# Autodesk Inventor assembly: 000-belt_liner_v1
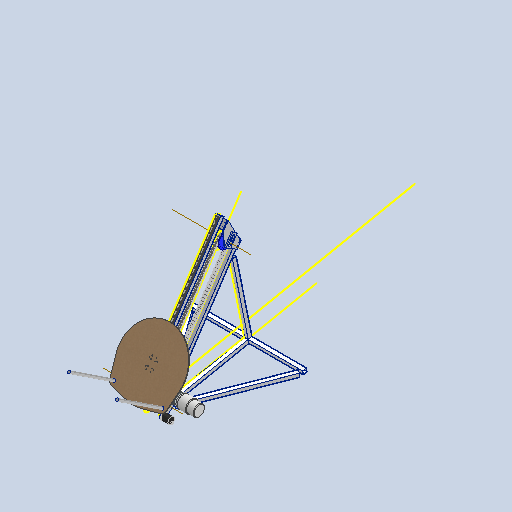
[picture p0: Inventor's stored thumbnail of the model, 512x512]
Saved by Autodesk Inventor 2025.1 (Build 291241000, 241)
## iProperties
Created: 2024-12-08
Part Number: 000-belt_liner_v1
Document SubType Name: Assembly
Designer: haruy
Author: haruy
## Documents named in this file (26)
- C:\Users\haruy\Documents\ロボコン\NHK2025\cad\nagahisa\belt_liner\000-belt_liner_v1.iam
- C:\Users\haruy\Documents\ロボコン\NHK2025\cad\nagahisa\belt_liner\belt_liner_v1_ASP_Base.ipt
- C:\Users\haruy\Documents\ロボコン\NHK2025\cad\nagahisa\belt_liner\SSE2B-MX10-455.iam
- C:\Users\haruy\Documents\ロボコン\NHK2025\cad\nagahisa\belt_liner\belt_liner_v1_Plate_1.ipt
- C:\Users\haruy\Documents\ロボコン\NHK2025\cad\nagahisa\belt_liner\belt_liner_v1_Plate_2.ipt
- C:\Users\haruy\Documents\ロボコン\NHK2025\cad\nagahisa\belt_liner\belt_liner_v1_Plate_3.ipt
- C:\Users\haruy\Documents\ロボコン\NHK2025\cad\000_parts\ベアリング\10\bear_10_15_sn.ipt
- C:\Users\haruy\Documents\ロボコン\NHK2025\cad\nagahisa\belt_liner\belt_liner_v1_shaft_spesa-25.ipt
- C:\Users\haruy\Documents\ロボコン\NHK2025\cad\nagahisa\belt_liner\belt_liner_v1_Plate_4.ipt
- C:\Users\haruy\Documents\ロボコン\NHK2025\cad\nagahisa\belt_liner\belt_liner_v1_Plate_5.ipt
- C:\Users\haruy\Documents\ロボコン\NHK2025\cad\000_parts\モーター\RS-775GM_004GH.iam
- C:\Users\haruy\Documents\ロボコン\NHK2025\cad\000_parts\エンコーダー\encoder v2.ipt
- C:\Users\haruy\Documents\ロボコン\NHK2025\cad\nagahisa\belt_liner\belt_liner_v1_Plate_6.ipt
- C:\Users\haruy\Documents\ロボコン\NHK2025\cad\nagahisa\belt_liner\belt_liner_v1_Plate_7.ipt
- C:\Users\haruy\Documents\ロボコン\NHK2025\cad\nagahisa\belt_liner\belt_liner_v1_Plate_8.ipt
- C:\Users\haruy\Documents\ロボコン\NHK2025\cad\nagahisa\belt_liner\belt_liner_v1_Plate_9.ipt
- C:\Users\haruy\Documents\ロボコン\NHK2025\cad\nagahisa\belt_liner\000-belt_liner_v1\デザイン アクセラレータ\歯付きベルト伝達1.iam
- C:\Users\haruy\Documents\ロボコン\NHK2025\cad\nagahisa\belt_liner\belt_liner_v1_shaft-54.ipt
- C:\Users\haruy\Documents\ロボコン\NHK2025\cad\nagahisa\belt_liner\SCSWJ10-6.iam
- C:\Users\haruy\Documents\ロボコン\NHK2025\cad\nagahisa\belt_liner\belt_liner_v1_shaft-84.ipt
- C:\Users\haruy\Documents\ロボコン\NHK2025\cad\nagahisa\belt_liner\000-belt_liner_v1\デザイン アクセラレータ\平歯車1.iam
- C:\Users\haruy\Documents\ロボコン\NHK2025\cad\nagahisa\belt_liner\000-belt_liner_v1\デザイン アクセラレータ\平歯車1_MIR.iam
- C:\Users\haruy\Documents\ロボコン\NHK2025\cad\nagahisa\belt_liner\belt_liner_v1_3DP_spesa-1.ipt
- C:\Users\haruy\Documents\ロボコン\NHK2025\cad\nagahisa\belt_liner\belt_liner_v1_3DP_spesa-2.ipt
- C:\Users\haruy\Documents\ロボコン\NHK2025\cad\nagahisa\belt_liner\belt_liner_v1_MDF_throw_plate.ipt
- C:\Users\haruy\Documents\ロボコン\NHK2025\cad\nagahisa\belt_liner\belt_liner_v1_shaft-200.ipt
## Components (44 placed, 25 different names)
1. belt_liner_v1_ASP_Base:1 — 挿入:1, 挿入:2, 挿入:3, 挿入:4, 挿入:5, 挿入:6, 挿入:28, 挿入:29, 挿入:30, 挿入:31, フラッシュ:1
2. SSE2B-MX10-455:1 [sub-assembly] — 挿入:1, 挿入:2, 挿入:51, 挿入:52
3. belt_liner_v1_Plate_1:1 — 挿入:3, 挿入:4
4. belt_liner_v1_Plate_2:1 — 挿入:5, 挿入:6, 挿入:7, 挿入:8, 挿入:9, 挿入:10
5. belt_liner_v1_Plate_3:1 — 挿入:7, 挿入:8, 挿入:12, 挿入:13, 挿入:14, 挿入:15, 挿入:16
6. belt_liner_v1_Plate_3:2 — 挿入:9, 挿入:10, 挿入:11, 挿入:19, 挿入:20, 挿入:21, 挿入:22
7. bear_10_15_sn:1 — 挿入:11
8. bear_10_15_sn:2 — 挿入:12, 挿入:50
9. belt_liner_v1_shaft_spesa-25:1 — 挿入:13, 挿入:17
10. belt_liner_v1_shaft_spesa-25:2 — 挿入:14, 挿入:18
11. belt_liner_v1_shaft_spesa-25:3 — 挿入:15
12. belt_liner_v1_shaft_spesa-25:4 — 挿入:16
13. belt_liner_v1_Plate_4:1 — 挿入:17, 挿入:18, 挿入:25, 挿入:27
14. belt_liner_v1_shaft_spesa-25:5 — 挿入:19, 挿入:24
15. belt_liner_v1_shaft_spesa-25:6 — 挿入:21
16. belt_liner_v1_shaft_spesa-25:7 — 挿入:20, 挿入:23
17. belt_liner_v1_shaft_spesa-25:8 — 挿入:22
18. belt_liner_v1_Plate_5:1 — 挿入:23, 挿入:24, 挿入:26
19. RS-775GM_004GH:1 [sub-assembly] — 挿入:25
20. RS-775GM_004GH:2 [sub-assembly] — 挿入:26, メイト:3
21. encoder v2:1 — 挿入:27
22. belt_liner_v1_Plate_6:1 — 挿入:28, 挿入:29, 挿入:32, 挿入:34, 挿入:35
23. belt_liner_v1_Plate_7:1 — 挿入:30, 挿入:31, 挿入:33
24. belt_liner_v1_Plate_8:1 — 挿入:32, 挿入:33, 挿入:36, 挿入:37
25. belt_liner_v1_Plate_8:2 — 挿入:34, 挿入:35, 挿入:38, 挿入:39
26. belt_liner_v1_Plate_9:1 — 挿入:38, 挿入:39
27. belt_liner_v1_Plate_9:2 — 挿入:36, 挿入:37
28. 歯付きベルト伝達:1 [sub-assembly] — 挿入:40, 挿入:41, 挿入:43, 挿入:49
29. bear_10_15_sn:3 — 挿入:40, 挿入:42, 挿入:47
30. bear_10_15_sn:4 — 挿入:41, 挿入:48
31. belt_liner_v1_shaft-54:1 — 挿入:42
32. SCSWJ10-6:1 [sub-assembly] — 挿入:43, 挿入:44
33. belt_liner_v1_shaft-84:1 — 挿入:44, 挿入:45, 挿入:46, メイト:1
34. SCSWJ10-6:2 [sub-assembly] — 挿入:45
35. SCSWJ10-6:3 [sub-assembly] — 挿入:46, メイト:2
36. 平歯車:1 [sub-assembly] — メイト:1, メイト:2, メイト:3
37. 平歯車1_MIR:1 [sub-assembly]
38. belt_liner_v1_3DP_spesa-1:1 — 挿入:47
39. belt_liner_v1_3DP_spesa-1:2 — 挿入:48
40. belt_liner_v1_3DP_spesa-1:3 — 挿入:49
41. belt_liner_v1_3DP_spesa-2:1 — 挿入:50
42. belt_liner_v1_MDF_throw_plate:1 — 挿入:51, 挿入:52, 挿入:53, 挿入:54
43. belt_liner_v1_shaft-200:1 — 挿入:54
44. belt_liner_v1_shaft-200:2 — 挿入:53
## Relationships (58: Insert 54, Mate 3, Flush 1)
- 挿入:1 [Insert]: belt_liner_v1_ASP_Base:1 ↔ SSE2B-MX10-455:1
- 挿入:2 [Insert]: belt_liner_v1_ASP_Base:1 ↔ SSE2B-MX10-455:1
- 挿入:3 [Insert]: belt_liner_v1_ASP_Base:1 ↔ belt_liner_v1_Plate_1:1
- 挿入:4 [Insert]: belt_liner_v1_ASP_Base:1 ↔ belt_liner_v1_Plate_1:1
- 挿入:5 [Insert]: belt_liner_v1_ASP_Base:1 ↔ belt_liner_v1_Plate_2:1
- 挿入:6 [Insert]: belt_liner_v1_ASP_Base:1 ↔ belt_liner_v1_Plate_2:1
- 挿入:7 [Insert]: belt_liner_v1_Plate_2:1 ↔ belt_liner_v1_Plate_3:1
- 挿入:8 [Insert]: belt_liner_v1_Plate_2:1 ↔ belt_liner_v1_Plate_3:1
- 挿入:9 [Insert]: belt_liner_v1_Plate_2:1 ↔ belt_liner_v1_Plate_3:2
- 挿入:10 [Insert]: belt_liner_v1_Plate_2:1 ↔ belt_liner_v1_Plate_3:2
- 挿入:11 [Insert]: belt_liner_v1_Plate_3:2 ↔ bear_10_15_sn:1
- 挿入:12 [Insert]: belt_liner_v1_Plate_3:1 ↔ bear_10_15_sn:2
- 挿入:13 [Insert]: belt_liner_v1_Plate_3:1 ↔ belt_liner_v1_shaft_spesa-25:1
- 挿入:14 [Insert]: belt_liner_v1_Plate_3:1 ↔ belt_liner_v1_shaft_spesa-25:2
- 挿入:15 [Insert]: belt_liner_v1_Plate_3:1 ↔ belt_liner_v1_shaft_spesa-25:3
- 挿入:16 [Insert]: belt_liner_v1_Plate_3:1 ↔ belt_liner_v1_shaft_spesa-25:4
- 挿入:17 [Insert]: belt_liner_v1_shaft_spesa-25:1 ↔ belt_liner_v1_Plate_4:1
- 挿入:18 [Insert]: belt_liner_v1_shaft_spesa-25:2 ↔ belt_liner_v1_Plate_4:1
- 挿入:19 [Insert]: belt_liner_v1_Plate_3:2 ↔ belt_liner_v1_shaft_spesa-25:5
- 挿入:20 [Insert]: belt_liner_v1_Plate_3:2 ↔ belt_liner_v1_shaft_spesa-25:7
- 挿入:21 [Insert]: belt_liner_v1_Plate_3:2 ↔ belt_liner_v1_shaft_spesa-25:6
- 挿入:22 [Insert]: belt_liner_v1_Plate_3:2 ↔ belt_liner_v1_shaft_spesa-25:8
- 挿入:23 [Insert]: belt_liner_v1_shaft_spesa-25:7 ↔ belt_liner_v1_Plate_5:1
- 挿入:24 [Insert]: belt_liner_v1_shaft_spesa-25:5 ↔ belt_liner_v1_Plate_5:1
- 挿入:25 [Insert]: belt_liner_v1_Plate_4:1 ↔ RS-775GM_004GH:1
- 挿入:26 [Insert]: belt_liner_v1_Plate_5:1 ↔ RS-775GM_004GH:2
- 挿入:27 [Insert]: belt_liner_v1_Plate_4:1 ↔ encoder v2:1
- 挿入:28 [Insert]: belt_liner_v1_ASP_Base:1 ↔ belt_liner_v1_Plate_6:1
- 挿入:29 [Insert]: belt_liner_v1_ASP_Base:1 ↔ belt_liner_v1_Plate_6:1
- 挿入:30 [Insert]: belt_liner_v1_ASP_Base:1 ↔ belt_liner_v1_Plate_7:1
- 挿入:31 [Insert]: belt_liner_v1_ASP_Base:1 ↔ belt_liner_v1_Plate_7:1
- 挿入:32 [Insert]: belt_liner_v1_Plate_6:1 ↔ belt_liner_v1_Plate_8:1
- 挿入:33 [Insert]: belt_liner_v1_Plate_7:1 ↔ belt_liner_v1_Plate_8:1
- 挿入:34 [Insert]: belt_liner_v1_Plate_6:1 ↔ belt_liner_v1_Plate_8:2
- 挿入:35 [Insert]: belt_liner_v1_Plate_6:1 ↔ belt_liner_v1_Plate_8:2
- 挿入:36 [Insert]: belt_liner_v1_Plate_8:1 ↔ belt_liner_v1_Plate_9:2
- 挿入:37 [Insert]: belt_liner_v1_Plate_8:1 ↔ belt_liner_v1_Plate_9:2
- 挿入:38 [Insert]: belt_liner_v1_Plate_8:2 ↔ belt_liner_v1_Plate_9:1
- 挿入:39 [Insert]: belt_liner_v1_Plate_8:2 ↔ belt_liner_v1_Plate_9:1
- フラッシュ:1 [Flush] (-7.5 mm): belt_liner_v1_ASP_Base:1
- 挿入:40 [Insert]: 歯付きベルト伝達:1 ↔ bear_10_15_sn:3
- 挿入:41 [Insert]: 歯付きベルト伝達:1 ↔ bear_10_15_sn:4
- 挿入:42 [Insert] (-16.5 mm): bear_10_15_sn:3 ↔ belt_liner_v1_shaft-54:1
- 挿入:43 [Insert]: 歯付きベルト伝達:1 ↔ SCSWJ10-6:1
- 挿入:44 [Insert] (-26.5 mm): SCSWJ10-6:1 ↔ belt_liner_v1_shaft-84:1
- 挿入:45 [Insert]: belt_liner_v1_shaft-84:1 ↔ SCSWJ10-6:2
- 挿入:46 [Insert]: belt_liner_v1_shaft-84:1 ↔ SCSWJ10-6:3
- メイト:1 [Mate]: belt_liner_v1_shaft-84:1 ↔ 平歯車:1
- メイト:2 [Mate]: SCSWJ10-6:3 ↔ 平歯車:1
- メイト:3 [Mate]: RS-775GM_004GH:2 ↔ 平歯車:1
- 挿入:47 [Insert]: bear_10_15_sn:3 ↔ belt_liner_v1_3DP_spesa-1:1
- 挿入:48 [Insert]: bear_10_15_sn:4 ↔ belt_liner_v1_3DP_spesa-1:2
- 挿入:49 [Insert]: 歯付きベルト伝達:1 ↔ belt_liner_v1_3DP_spesa-1:3
- 挿入:50 [Insert]: bear_10_15_sn:2 ↔ belt_liner_v1_3DP_spesa-2:1
- 挿入:51 [Insert]: SSE2B-MX10-455:1 ↔ belt_liner_v1_MDF_throw_plate:1
- 挿入:52 [Insert]: SSE2B-MX10-455:1 ↔ belt_liner_v1_MDF_throw_plate:1
- 挿入:53 [Insert]: belt_liner_v1_MDF_throw_plate:1 ↔ belt_liner_v1_shaft-200:2
- 挿入:54 [Insert]: belt_liner_v1_MDF_throw_plate:1 ↔ belt_liner_v1_shaft-200:1
